# Autodesk Inventor assembly: 조립품1
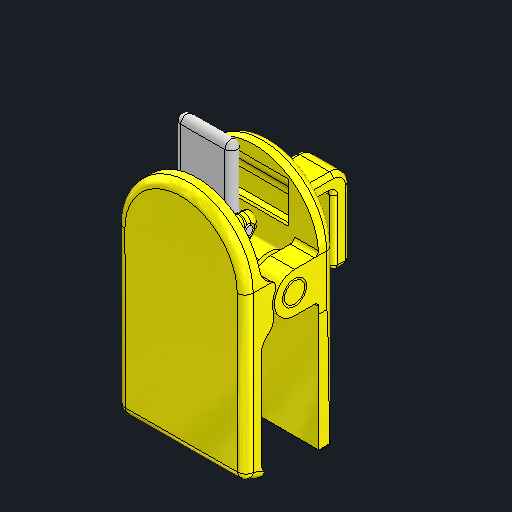
[picture p0: Inventor's stored thumbnail of the model, 512x512]
Saved by Autodesk Inventor 2024.1 (Build 281209000, 209)
## iProperties
Created: 2024-01-27
Part Number: 조립품1
Document SubType Name: Assembly
Designer: likek
Author: likek
## Documents named in this file (4)
- C:\Users\likek\Videos\Modeling\IKEA 페그보드 시제품\Peg\SKÅDIS Pegboard Peg.iam
- C:\Users\likek\Videos\Modeling\IKEA 페그보드 시제품\Peg\1-1.ipt
- C:\Users\likek\Videos\Modeling\IKEA 페그보드 시제품\Peg\1-2.ipt
- C:\Users\likek\Videos\Modeling\IKEA 페그보드 시제품\Peg\1-3.ipt
## Components (3 placed, 3 different names)
1. 1-1:1 — 삽입:1, 각도:2
2. 1-2:1 — 삽입:1, 각도:2, 삽입:2
3. 1-3:1 — 삽입:2
## Relationships (3: Insert 2, Angle 1)
- 삽입:1 [Insert]: 1-1:1 ↔ 1-2:1
- 각도:2 [Angle] (180 deg): 1-1:1 ↔ 1-2:1
- 삽입:2 [Insert]: 1-2:1 ↔ 1-3:1
